# Autodesk Inventor assembly: сборка акб
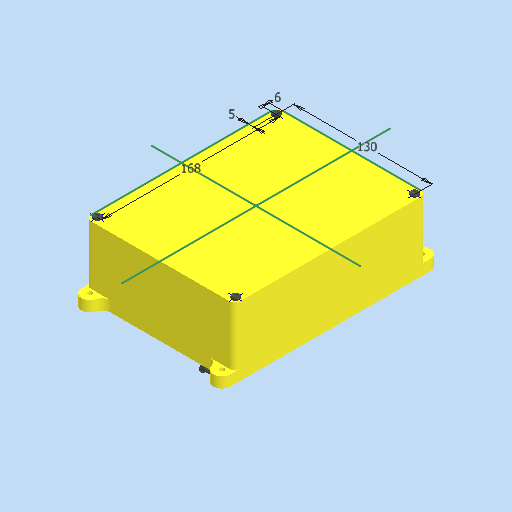
[picture p0: Inventor's stored thumbnail of the model, 512x512]
Saved by Autodesk Inventor 2025 (Build 290162000, 162)
## iProperties
Created: 2025-02-26
Part Number: сборка акб
Document SubType Name: Assembly
Designer: volko
Mass: 2301.02 g
Surface Area: 2393.18 cm^2
Volume: 1376.28 cm^3
Density: 1.67192 g/cm^3
Author: volko
## Documents named in this file (6)
- C:\Users\volko\Desktop\диплом\Модели\детали\сборка акб.iam
- C:\Users\volko\Desktop\диплом\Модели\детали\акб корпус.ipt
- C:\Users\volko\Desktop\диплом\Модели\детали\акб.ipt
- C:\Users\volko\Desktop\диплом\Модели\детали\акб_MIR.ipt
- C:\Users\volko\Desktop\диплом\Модели\детали\крышка акб.ipt
- C:\Users\volko\Desktop\диплом\Модели\детали\стандартные изделия\ru-RU\ISO 7380-1\ISO 7380-1 - M4 x 10.ipt
## Components (9 placed, 5 different names)
1. акб корпус:1 — Заподлицо:1, Заподлицо:2, Заподлицо:3, Совмещение:1, Заподлицо:4, Совмещение:2, Совмещение:3, Совмещение:6, Совмещение:7
2. акб:1 — Совмещение:1, Заподлицо:4, Совмещение:2, Симметрия:1
3. акб_MIR:1 — Симметрия:1, Совмещение:3, Совмещение:4
4. крышка акб:1 — Совмещение:5, Совмещение:6, Заподлицо:5, Совмещение:8
5. ISO 7380-1 M4 x 10:1
6. ISO 7380-1 M4 x 10:2 — Совмещение:7, Совмещение:8
7. ISO 7380-1 M4 x 10:3
8. ISO 7380-1 M4 x 10:4
9. ISO 7380-1 M4 x 10:5
## Component patterns: (4 elements, first: ISO 7380-1 M4 x 10:2)
## Relationships (14: Mate 8, Flush 5, Symmetry 1)
- Заподлицо:1 [Flush]: акб корпус:1
- Заподлицо:2 [Flush]: акб корпус:1
- Заподлицо:3 [Flush]: акб корпус:1
- Совмещение:1 [Mate]: акб корпус:1 ↔ акб:1
- Заподлицо:4 [Flush]: акб корпус:1 ↔ акб:1
- Совмещение:2 [Mate] (3.5 mm): акб корпус:1 ↔ акб:1
- Симметрия:1 [Symmetry]: акб:1 ↔ акб_MIR:1
- Совмещение:3 [Mate]: акб корпус:1 ↔ акб_MIR:1
- Совмещение:4 [Mate]: акб_MIR:1
- Совмещение:5 [Mate]: крышка акб:1
- Совмещение:6 [Mate]: акб корпус:1 ↔ крышка акб:1
- Заподлицо:5 [Flush]: крышка акб:1
- Совмещение:7 [Mate]: акб корпус:1 ↔ ISO 7380-1 M4 x 10:2
- Совмещение:8 [Mate]: крышка акб:1 ↔ ISO 7380-1 M4 x 10:2
